# Autodesk Inventor assembly: СОВЕРШЕНСТВО
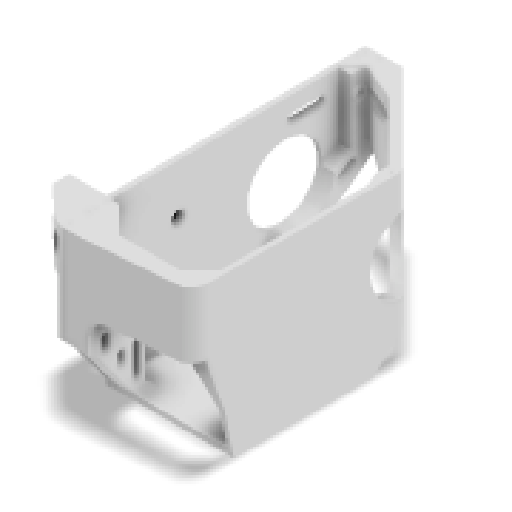
[picture p0: Inventor's stored thumbnail of the model, 512x512]
Saved by Autodesk Inventor 2025 (Build 290162000, 162)
## iProperties
Created: 2024-10-08
Part Number: СОВЕРШЕНСТВО
Document SubType Name: Assembly
Designer: Phantom
Mass: 291.072 g
Surface Area: 978.884 cm^2
Volume: 188.885 cm^3
Density: 1.541 g/cm^3
Author: Phantom
## Documents named in this file (10)
- C:\Users\GameHD\Desktop\phantom 16950\СОВЕРШЕНСТВО без говна.iam
- C:\Users\GameHD\Desktop\phantom 16950\репление колёс СОВЕРШЕННОЕ ТОЛСТАЯ.ipt
- C:\Users\GameHD\Desktop\phantom 16950\репление колёс СОВЕРШЕННОЕ ТОНКАЯ.ipt
- C:\Users\GameHD\Desktop\phantom 16950\СОВЕРШЕНСТВО без говна\AIP\FEA\eyixam7a9.fres
- C:\Users\GameHD\Desktop\phantom 16950\СОВЕРШЕНСТВО без говна\AIP\FEA\eyixam79c.fins
- C:\Users\GameHD\Desktop\phantom 16950\СОВЕРШЕНСТВО без говна\AIP\FEA\eyixam79c.fsat
- C:\Users\GameHD\Desktop\phantom 16950\СОВЕРШЕНСТВО без говна\AIP\FEA\eyixam79c.ftes
- C:\Users\GameHD\Desktop\phantom 16950\СОВЕРШЕНСТВО без говна\AIP\FEA\eyixam79c.fwiz
- C:\Users\GameHD\Desktop\phantom 16950\СОВЕРШЕНСТВО без говна\AIP\FEA\eyixam7a8.fmsh
- C:\Users\GameHD\Desktop\phantom 16950\СОВЕРШЕНСТВО без говна\AIP\FEA\eyj0cf4qo.fres
## Components (2 placed, 2 different names)
1. репление колёс СОВЕРШЕННОЕ ТОЛСТАЯ:1 — Совмещение:1, Заподлицо:1, Совмещение:2
2. репление колёс СОВЕРШЕННОЕ ТОНКАЯ:1 — Совмещение:1, Заподлицо:1, Совмещение:2
## Relationships (3: Mate 2, Flush 1)
- Совмещение:1 [Mate]: репление колёс СОВЕРШЕННОЕ ТОЛСТАЯ:1 ↔ репление колёс СОВЕРШЕННОЕ ТОНКАЯ:1
- Заподлицо:1 [Flush]: репление колёс СОВЕРШЕННОЕ ТОЛСТАЯ:1 ↔ репление колёс СОВЕРШЕННОЕ ТОНКАЯ:1
- Совмещение:2 [Mate]: репление колёс СОВЕРШЕННОЕ ТОЛСТАЯ:1 ↔ репление колёс СОВЕРШЕННОЕ ТОНКАЯ:1
## Named parameters: sa_0 = 20000, sa_1 = 20000
note: some values were not read from the file. Shown as the stored number, unit unknown: "sa_0", "sa_1".
